# Autodesk Inventor assembly: Rama_wozka
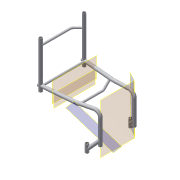
[picture p0: Inventor's stored thumbnail of the model, 180x180]
Saved by Autodesk Inventor 2015 (Build 190159000, 159)
## iProperties
Created: 2015-11-22
Part Number: Rama_wozka
Document SubType Name: Weldment
Designer: graaapsik
Weld Material: Aluminium AW-7020
Author: graaapsik
## Documents named in this file (3)
- C:\Users\EriveltonDell\Documents\Centro Universitário da FEI\Wheelchair\CADEIRA DE RODAS - DESENHO\Model\Rama_wozka.iam
- C:\Users\EriveltonDell\Documents\Centro Universitário da FEI\Wheelchair\CADEIRA DE RODAS - DESENHO\Model\Rama_oparcia.iam
- C:\Users\EriveltonDell\Documents\Centro Universitário da FEI\Wheelchair\CADEIRA DE RODAS - DESENHO\Model\Rama_siedziska.iam
## Components (2 placed, 2 different names)
1. Rama_siedziska:1 [sub-assembly] — Zestawiający:1, Zestawiający:2, Równoległy:1, Zestawiający:3, Zestawiający:4
2. Rama_oparcia:1 [sub-assembly] — Zestawiający:1, Zestawiający:2, Równoległy:1
## Relationships (7: Mate 6, Flush 1)
- Zestawiający:1 [Mate] (-20 mm): Rama_siedziska:1 ↔ Rama_oparcia:1
- Zestawiający:2 [Mate] (-50 mm): Rama_siedziska:1 ↔ Rama_oparcia:1
- Równoległy:1 [Flush] (16 mm): Rama_siedziska:1 ↔ Rama_oparcia:1
- Zestawiający:3 [Mate]: Rama_siedziska:1
- Zestawiający:4 [Mate]: Rama_siedziska:1
- Zestawiający:5 [Mate]
- Zestawiający:6 [Mate]
